# Autodesk Inventor assembly: PalaVerticala
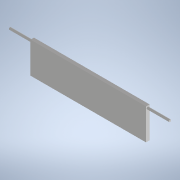
[picture p0: Inventor's stored thumbnail of the model, 180x180]
Saved by Autodesk Inventor 2020.3 (Build 243373000, 373)
## iProperties
Created: 2021-03-20
Part Number: PalaVerticala
Document SubType Name: Assembly
Designer: alexo
Author: alexo
## Documents named in this file (3)
- C:\Users\alexo\Documents\Inventor\TheArch\R&D\Beta0\Structura\Motor\PalaVerticala.iam
- C:\Users\alexo\Documents\Inventor\TheArch\R&D\Beta0\Structura\Motor\Pala.ipt
- C:\Users\alexo\Documents\Inventor\TheArch\R&D\Beta0\Structura\Extra\TijaAluminiu2.5x180.ipt
## Components (2 placed, 2 different names)
1. Pala:1 — Rigid:1
2. TijaAluminiu2.5x180:1 — Rigid:1
## Relationships (1: WeldJoint 1)
- Rigid:1 [WeldJoint]: Pala:1 ↔ TijaAluminiu2.5x180:1
